# Autodesk Inventor assembly: 知能ロボットver2
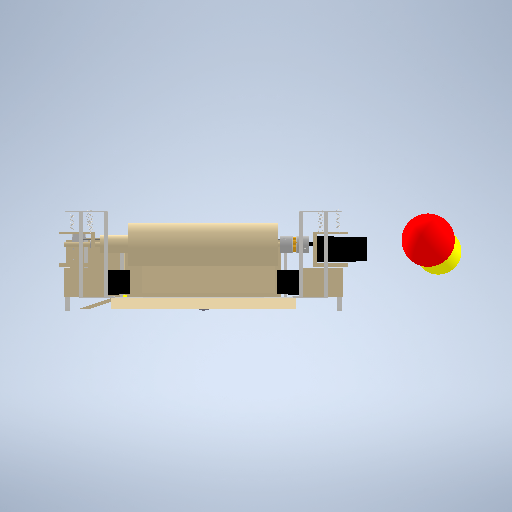
[picture p0: Inventor's stored thumbnail of the model, 512x512]
Saved by Autodesk Inventor 2026.2 (Build 302298010, 298A)
## iProperties
Created: 2026-05-06
Part Number: 知能ロボットver2
Document SubType Name: Assembly
Designer: Yagis
Author: Yagis
## Documents named in this file (34)
- C:\Users\Yagis\OneDrive\ドキュメント\知能ロボット\知能ロボットver2.iam
- C:\Users\Yagis\OneDrive\ドキュメント\知能ロボット\L-Bracket.ipt
- C:\Users\Yagis\OneDrive\ドキュメント\知能ロボット\Metal Gearmotor.ipt
- C:\Users\Yagis\OneDrive\ドキュメント\知能ロボット\タイヤ.ipt
- C:\Users\Yagis\OneDrive\ドキュメント\知能ロボット\キャスタ420G-R32.ipt
- C:\Users\Yagis\OneDrive\ドキュメント\知能ロボット\知能ロボ土台.ipt
- C:\Users\Yagis\OneDrive\ドキュメント\知能ロボット\キャスター土台.ipt
- C:\Users\Yagis\OneDrive\ドキュメント\知能ロボット\キャスタスペーサ.ipt
- C:\Users\Yagis\OneDrive\ドキュメント\知能ロボット\ラインセンサ.ipt
- C:\Users\Yagis\OneDrive\ドキュメント\知能ロボット\ライントレーズスペーサ.ipt
- C:\Users\Yagis\OneDrive\ドキュメント\知能ロボット\ボール.ipt
- C:\Users\Yagis\OneDrive\ドキュメント\知能ロボット\ボール2.ipt
- C:\Users\Yagis\OneDrive\ドキュメント\知能ロボット\回収機構スペーサ.ipt
- C:\Users\Yagis\OneDrive\ドキュメント\知能ロボット\回収機構天井.ipt
- C:\Users\Yagis\OneDrive\ドキュメント\知能ロボット\ギアボックス.ipt
- C:\Users\Yagis\OneDrive\ドキュメント\知能ロボット\ギアボックス2.ipt
- C:\Users\Yagis\OneDrive\ドキュメント\知能ロボット\C-FL678ZZ.ipt
- C:\Users\Yagis\OneDrive\ドキュメント\知能ロボット\天板.ipt
- C:\Users\Yagis\OneDrive\ドキュメント\知能ロボット\天板スペーサ.ipt
- C:\Users\Yagis\OneDrive\ドキュメント\知能ロボット\自作ローラ.ipt
- C:\Users\Yagis\OneDrive\ドキュメント\知能ロボット\排出機構.ipt
- C:\Users\Yagis\OneDrive\ドキュメント\知能ロボット\左仕切り.ipt
- C:\Users\Yagis\OneDrive\ドキュメント\知能ロボット\右仕切り.ipt
- C:\Users\Yagis\OneDrive\ドキュメント\知能ロボット\MSF-25 - 6-8 Casing 2.ipt
- C:\Users\Yagis\OneDrive\ドキュメント\知能ロボット\MSF-25 Sleeve.ipt
- C:\Users\Yagis\OneDrive\ドキュメント\知能ロボット\MSF-25 - 6-8 Casing 1.ipt
- C:\Users\Yagis\OneDrive\ドキュメント\知能ロボット\サーボパーツ2.ipt
- C:\Users\Yagis\OneDrive\ドキュメント\知能ロボット\サーボパーツ1.ipt
- C:\Users\Yagis\OneDrive\ドキュメント\知能ロボット\バンパー2.ipt
- C:\Users\Yagis\OneDrive\ドキュメント\知能ロボット\バンパー1.ipt
- C:\Users\Yagis\OneDrive\ドキュメント\知能ロボット\排出スロープ.ipt
- C:\Users\Yagis\OneDrive\ドキュメント\知能ロボット\引張りコイルばね11.ipt
- C:\Users\Yagis\OneDrive\ドキュメント\知能ロボット\モータ土台.ipt
- C:\Users\Yagis\OneDrive\ドキュメント\知能ロボット\坂.ipt
## Components (61 placed, 33 different names)
1. L-Bracket:1 — 挿入:9, 挿入:10, 挿入:11, 挿入:12, 挿入:13, 挿入:14, 挿入:25, 挿入:26, 挿入:27, 挿入:28
2. L-Bracket:2 — 挿入:15, 挿入:16, 挿入:17, 挿入:18, 挿入:19, 挿入:20, 挿入:23, 挿入:24, 挿入:29, 挿入:30
3. Metal Gearmotor:1 — 挿入:9, 挿入:10, 挿入:11, 挿入:12, 挿入:13, 挿入:14, 挿入:21
4. Metal Gearmotor:2 — 挿入:15, 挿入:16, 挿入:17, 挿入:18, 挿入:19, 挿入:20, 挿入:22
5. タイヤ:1 — 挿入:21
6. タイヤ:2 — 挿入:22
7. キャスタ420G-R32:1 — 挿入:35, 挿入:36, 挿入:37, 挿入:38
8. 知能ロボ土台:1 — 挿入:23, 挿入:24, 挿入:25, 挿入:26, 挿入:27, 挿入:28, 挿入:29, 挿入:30, 挿入:39, 挿入:41, 挿入:43, 挿入:45, 挿入:47, 挿入:49, 挿入:55, 挿入:56, 挿入:57, 挿入:58, 挿入:59, 挿入:60, 挿入:61, 挿入:62, 角度:12, 角度:13, 挿入:98, 挿入:99, 挿入:100, 挿入:101, 角度:14, 角度:17, 挿入:112, 挿入:129, 挿入:130, 挿入:131, 挿入:132, 挿入:133, 挿入:134, 挿入:137, 挿入:138, 挿入:139, 挿入:140, 挿入:141, 挿入:142, 挿入:143, 挿入:144
9. キャスター土台:1 — 挿入:35, 挿入:36, 挿入:37, 挿入:38, 挿入:40, 挿入:42, 挿入:44, 挿入:46
10. キャスタスペーサ:1 — 挿入:39, 挿入:40
11. キャスタスペーサ:2 — 挿入:41, 挿入:42
12. キャスタスペーサ:3 — 挿入:43, 挿入:44
13. キャスタスペーサ:4 — 挿入:45, 挿入:46
14. ラインセンサ:1 — 挿入:48, 挿入:50
15. ライントレーズスペーサ:1 — 挿入:49, 挿入:50
16. ライントレーズスペーサ:2 — 挿入:47, 挿入:48
17. ボール:1
18. ボール2:1
19. 回収機構スペーサ:1 — 挿入:57, 挿入:67, 角度:5, 角度:7, 角度:8, 角度:12
20. 回収機構スペーサ:2 — 挿入:58, 挿入:65, 角度:7
21. 回収機構スペーサ:3 — 挿入:55, 挿入:66, 角度:6
22. 回収機構スペーサ:4 — 挿入:56, 挿入:68, 角度:5, 角度:6
23. 回収機構スペーサ:5 — 挿入:60, 角度:2, 挿入:87
24. 回収機構スペーサ:6 — 挿入:62, 角度:4, 挿入:89, 角度:10, 角度:13
25. 回収機構スペーサ:7 — 挿入:61, 角度:3, 角度:4, 挿入:86
26. 回収機構スペーサ:8 — 挿入:59, 角度:2, 角度:3, 挿入:88
27. 回収機構天井:1 — 挿入:65, 挿入:66, 挿入:67, 挿入:68, 角度:9
28. 回収機構天井:2 — 挿入:86, 挿入:87, 挿入:88, 挿入:89, 角度:11
29. Metal Gearmotor:3 — 挿入:79, 挿入:80, 挿入:81, 挿入:82, 挿入:83, 挿入:84, 挿入:119
30. ギアボックス:1 — 挿入:79, 挿入:80, 挿入:81, 挿入:82, 挿入:83, 挿入:84, 角度:8, 角度:9
31. ギアボックス2:1 — 挿入:94, 角度:10, 角度:11
32. C-FL678ZZ:1 — 挿入:94, 挿入:121
33. 天板:1 — 挿入:108, 挿入:109, 挿入:110, 挿入:111, 挿入:113, 挿入:114, 挿入:115, 挿入:116, 挿入:117, 挿入:118
34. 天板スペーサ:1 — 挿入:98, 角度:15, 挿入:110
35. 天板スペーサ:2 — 挿入:99, 角度:14, 角度:15, 挿入:111
36. 天板スペーサ:3 — 挿入:101, 角度:16, 角度:17, 挿入:109
37. 天板スペーサ:4 — 挿入:100, 角度:16, 挿入:108
38. 自作ローラ:1 — 挿入:120, 挿入:121
39. 排出機構:1 — 挿入:135, 挿入:136
40. 天板スペーサ:5 — 挿入:112, 挿入:113
41. 左仕切り:1 — 挿入:114, 挿入:115, 挿入:123, 挿入:124, 挿入:125, 挿入:126, 挿入:127, 挿入:128
42. 右仕切り:1 — 挿入:116, 挿入:117, 挿入:118
43. MSF-25 - 6-8 Casing 2:1 — 回転:4, 挿入:120
44. MSF-25 Sleeve:1 — 回転:3, 回転:4
45. MSF-25 - 6-8 Casing 1:1 — 回転:3, 挿入:119
46. サーボパーツ2:1 — 挿入:122, 挿入:135, 挿入:136
47. サーボパーツ1:1 — 挿入:122, 挿入:123, 挿入:124, 挿入:125, 挿入:126, 挿入:127, 挿入:128
48. バンパー2:1 — 挿入:129, 挿入:130
49. バンパー1:1 — 挿入:131, 挿入:132
50. 排出スロープ:1 — 挿入:133, 挿入:134
51. 引張りコイルばね1:1
52. 引張りコイルばね1:2
53. 引張りコイルばね1:8
54. 引張りコイルばね1:9
55. 引張りコイルばね1:10
56. 引張りコイルばね1:14
57. 引張りコイルばね1:15
58. 引張りコイルばね1:16
59. モータ土台:1 — 挿入:141, 挿入:142, 挿入:143, 挿入:144
60. モータ土台:2 — 挿入:137, 挿入:138, 挿入:139, 挿入:140
61. 坂:1
## Relationships (120: Insert 102, Angle 16, RevoluteJoint 2)
- 挿入:9 [Insert]: L-Bracket:1 ↔ Metal Gearmotor:1
- 挿入:10 [Insert]: L-Bracket:1 ↔ Metal Gearmotor:1
- 挿入:11 [Insert]: L-Bracket:1 ↔ Metal Gearmotor:1
- 挿入:12 [Insert]: L-Bracket:1 ↔ Metal Gearmotor:1
- 挿入:13 [Insert]: L-Bracket:1 ↔ Metal Gearmotor:1
- 挿入:14 [Insert]: L-Bracket:1 ↔ Metal Gearmotor:1
- 挿入:15 [Insert]: L-Bracket:2 ↔ Metal Gearmotor:2
- 挿入:16 [Insert]: L-Bracket:2 ↔ Metal Gearmotor:2
- 挿入:17 [Insert]: L-Bracket:2 ↔ Metal Gearmotor:2
- 挿入:18 [Insert]: L-Bracket:2 ↔ Metal Gearmotor:2
- 挿入:19 [Insert]: L-Bracket:2 ↔ Metal Gearmotor:2
- 挿入:20 [Insert]: L-Bracket:2 ↔ Metal Gearmotor:2
- 挿入:21 [Insert]: Metal Gearmotor:1 ↔ タイヤ:1
- 挿入:22 [Insert]: Metal Gearmotor:2 ↔ タイヤ:2
- 挿入:23 [Insert]: L-Bracket:2 ↔ 知能ロボ土台:1
- 挿入:24 [Insert]: L-Bracket:2 ↔ 知能ロボ土台:1
- 挿入:25 [Insert]: L-Bracket:1 ↔ 知能ロボ土台:1
- 挿入:26 [Insert]: L-Bracket:1 ↔ 知能ロボ土台:1
- 挿入:27 [Insert]: L-Bracket:1 ↔ 知能ロボ土台:1
- 挿入:28 [Insert]: L-Bracket:1 ↔ 知能ロボ土台:1
- 挿入:29 [Insert]: L-Bracket:2 ↔ 知能ロボ土台:1
- 挿入:30 [Insert]: L-Bracket:2 ↔ 知能ロボ土台:1
- 挿入:35 [Insert]: キャスタ420G-R32:1 ↔ キャスター土台:1
- 挿入:36 [Insert]: キャスタ420G-R32:1 ↔ キャスター土台:1
- 挿入:37 [Insert]: キャスタ420G-R32:1 ↔ キャスター土台:1
- 挿入:38 [Insert]: キャスタ420G-R32:1 ↔ キャスター土台:1
- 挿入:39 [Insert]: 知能ロボ土台:1 ↔ キャスタスペーサ:1
- 挿入:40 [Insert]: キャスター土台:1 ↔ キャスタスペーサ:1
- 挿入:41 [Insert]: 知能ロボ土台:1 ↔ キャスタスペーサ:2
- 挿入:42 [Insert]: キャスター土台:1 ↔ キャスタスペーサ:2
- 挿入:43 [Insert]: 知能ロボ土台:1 ↔ キャスタスペーサ:3
- 挿入:44 [Insert]: キャスター土台:1 ↔ キャスタスペーサ:3
- 挿入:45 [Insert]: 知能ロボ土台:1 ↔ キャスタスペーサ:4
- 挿入:46 [Insert]: キャスター土台:1 ↔ キャスタスペーサ:4
- 挿入:47 [Insert]: 知能ロボ土台:1 ↔ ライントレーズスペーサ:2
- 挿入:48 [Insert]: ラインセンサ:1 ↔ ライントレーズスペーサ:2
- 挿入:49 [Insert]: 知能ロボ土台:1 ↔ ライントレーズスペーサ:1
- 挿入:50 [Insert]: ラインセンサ:1 ↔ ライントレーズスペーサ:1
- 挿入:55 [Insert]: 知能ロボ土台:1 ↔ 回収機構スペーサ:3
- 挿入:56 [Insert]: 知能ロボ土台:1 ↔ 回収機構スペーサ:4
- 挿入:57 [Insert]: 知能ロボ土台:1 ↔ 回収機構スペーサ:1
- 挿入:58 [Insert]: 知能ロボ土台:1 ↔ 回収機構スペーサ:2
- 挿入:59 [Insert]: 知能ロボ土台:1 ↔ 回収機構スペーサ:8
- 挿入:60 [Insert]: 知能ロボ土台:1 ↔ 回収機構スペーサ:5
- 挿入:61 [Insert]: 知能ロボ土台:1 ↔ 回収機構スペーサ:7
- 挿入:62 [Insert]: 知能ロボ土台:1 ↔ 回収機構スペーサ:6
- 挿入:65 [Insert]: 回収機構スペーサ:2 ↔ 回収機構天井:1
- 挿入:66 [Insert]: 回収機構スペーサ:3 ↔ 回収機構天井:1
- 挿入:67 [Insert]: 回収機構スペーサ:1 ↔ 回収機構天井:1
- 挿入:68 [Insert]: 回収機構スペーサ:4 ↔ 回収機構天井:1
- 挿入:79 [Insert]: Metal Gearmotor:3 ↔ ギアボックス:1
- 挿入:80 [Insert]: Metal Gearmotor:3 ↔ ギアボックス:1
- 挿入:81 [Insert]: Metal Gearmotor:3 ↔ ギアボックス:1
- 挿入:82 [Insert]: Metal Gearmotor:3 ↔ ギアボックス:1
- 挿入:83 [Insert]: Metal Gearmotor:3 ↔ ギアボックス:1
- 挿入:84 [Insert]: Metal Gearmotor:3 ↔ ギアボックス:1
- 角度:2 [Angle] (0 deg): 回収機構スペーサ:5 ↔ 回収機構スペーサ:8
- 角度:3 [Angle] (0 deg): 回収機構スペーサ:7 ↔ 回収機構スペーサ:8
- 角度:4 [Angle] (0 deg): 回収機構スペーサ:6 ↔ 回収機構スペーサ:7
- 角度:5 [Angle] (0 deg): 回収機構スペーサ:1 ↔ 回収機構スペーサ:4
- 角度:6 [Angle] (0 deg): 回収機構スペーサ:3 ↔ 回収機構スペーサ:4
- 角度:7 [Angle] (0 deg): 回収機構スペーサ:1 ↔ 回収機構スペーサ:2
- 挿入:86 [Insert]: 回収機構スペーサ:7 ↔ 回収機構天井:2
- 挿入:87 [Insert]: 回収機構スペーサ:5 ↔ 回収機構天井:2
- 挿入:88 [Insert]: 回収機構スペーサ:8 ↔ 回収機構天井:2
- 挿入:89 [Insert]: 回収機構スペーサ:6 ↔ 回収機構天井:2
- 挿入:94 [Insert]: ギアボックス2:1 ↔ C-FL678ZZ:1
- 角度:8 [Angle] (0 deg): 回収機構スペーサ:1 ↔ ギアボックス:1
- 角度:9 [Angle] (0 deg): 回収機構天井:1 ↔ ギアボックス:1
- 角度:10 [Angle] (0 deg): 回収機構スペーサ:6 ↔ ギアボックス2:1
- 角度:11 [Angle] (0 deg): 回収機構天井:2 ↔ ギアボックス2:1
- 角度:12 [Angle] (0 deg): 知能ロボ土台:1 ↔ 回収機構スペーサ:1
- 角度:13 [Angle] (0 deg): 知能ロボ土台:1 ↔ 回収機構スペーサ:6
- 挿入:98 [Insert]: 知能ロボ土台:1 ↔ 天板スペーサ:1
- 挿入:99 [Insert]: 知能ロボ土台:1 ↔ 天板スペーサ:2
- 挿入:100 [Insert]: 知能ロボ土台:1 ↔ 天板スペーサ:4
- 挿入:101 [Insert]: 知能ロボ土台:1 ↔ 天板スペーサ:3
- 角度:14 [Angle] (0 deg): 知能ロボ土台:1 ↔ 天板スペーサ:2
- 角度:15 [Angle] (0 deg): 天板スペーサ:1 ↔ 天板スペーサ:2
- 角度:16 [Angle] (0 deg): 天板スペーサ:3 ↔ 天板スペーサ:4
- 角度:17 [Angle] (0 deg): 知能ロボ土台:1 ↔ 天板スペーサ:3
- 挿入:108 [Insert]: 天板:1 ↔ 天板スペーサ:4
- 挿入:109 [Insert]: 天板:1 ↔ 天板スペーサ:3
- 挿入:110 [Insert]: 天板:1 ↔ 天板スペーサ:1
- 挿入:111 [Insert]: 天板:1 ↔ 天板スペーサ:2
- 挿入:112 [Insert]: 知能ロボ土台:1 ↔ 天板スペーサ:5
- 挿入:113 [Insert]: 天板:1 ↔ 天板スペーサ:5
- 挿入:114 [Insert]: 天板:1 ↔ 左仕切り:1
- 挿入:115 [Insert]: 天板:1 ↔ 左仕切り:1
- 挿入:116 [Insert]: 天板:1 ↔ 右仕切り:1
- 挿入:117 [Insert]: 天板:1 ↔ 右仕切り:1
- 挿入:118 [Insert]: 天板:1 ↔ 右仕切り:1
- 回転:3 [RevoluteJoint]: MSF-25 Sleeve:1 ↔ MSF-25 - 6-8 Casing 1:1
- 回転:4 [RevoluteJoint]: MSF-25 - 6-8 Casing 2:1 ↔ MSF-25 Sleeve:1
- 挿入:119 [Insert] (-11 mm): Metal Gearmotor:3 ↔ MSF-25 - 6-8 Casing 1:1
- 挿入:120 [Insert] (-9 mm): 自作ローラ:1 ↔ MSF-25 - 6-8 Casing 2:1
- 挿入:121 [Insert] (36 mm): C-FL678ZZ:1 ↔ 自作ローラ:1
- 挿入:122 [Insert] (2 mm): サーボパーツ2:1 ↔ サーボパーツ1:1
- 挿入:123 [Insert]: 左仕切り:1 ↔ サーボパーツ1:1
- 挿入:124 [Insert]: 左仕切り:1 ↔ サーボパーツ1:1
- 挿入:125 [Insert] (0.5 mm): 左仕切り:1 ↔ サーボパーツ1:1
- 挿入:126 [Insert] (0.5 mm): 左仕切り:1 ↔ サーボパーツ1:1
- 挿入:127 [Insert] (0.5 mm): 左仕切り:1 ↔ サーボパーツ1:1
- 挿入:128 [Insert] (0.5 mm): 左仕切り:1 ↔ サーボパーツ1:1
- 挿入:129 [Insert]: 知能ロボ土台:1 ↔ バンパー2:1
- 挿入:130 [Insert]: 知能ロボ土台:1 ↔ バンパー2:1
- 挿入:131 [Insert]: 知能ロボ土台:1 ↔ バンパー1:1
- 挿入:132 [Insert]: 知能ロボ土台:1 ↔ バンパー1:1
- 挿入:133 [Insert]: 知能ロボ土台:1 ↔ 排出スロープ:1
- 挿入:134 [Insert]: 知能ロボ土台:1 ↔ 排出スロープ:1
- 挿入:135 [Insert]: 排出機構:1 ↔ サーボパーツ2:1
- 挿入:136 [Insert]: 排出機構:1 ↔ サーボパーツ2:1
- 挿入:137 [Insert]: 知能ロボ土台:1 ↔ モータ土台:2
- 挿入:138 [Insert]: 知能ロボ土台:1 ↔ モータ土台:2
- 挿入:139 [Insert]: 知能ロボ土台:1 ↔ モータ土台:2
- 挿入:140 [Insert]: 知能ロボ土台:1 ↔ モータ土台:2
- 挿入:141 [Insert]: 知能ロボ土台:1 ↔ モータ土台:1
- 挿入:142 [Insert]: 知能ロボ土台:1 ↔ モータ土台:1
- 挿入:143 [Insert]: 知能ロボ土台:1 ↔ モータ土台:1
- 挿入:144 [Insert]: 知能ロボ土台:1 ↔ モータ土台:1
## Named parameters: Finish1_Area = 2226.12, Finish1_Thickness = 0.05 mm, Finish2_Area = 2918.95, Finish2_Thickness = 0.05 mm, Finish3_Area = 2892.68, Finish3_Thickness = 0.05 mm
note: some values were not read from the file. Shown as the stored number, unit unknown: "Finish1_Area", "Finish2_Area", "Finish3_Area".
